# Autodesk Inventor assembly: Assembly_final
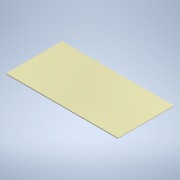
[picture p0: Inventor's stored thumbnail of the model, 180x180]
Saved by Autodesk Inventor 2021 (Build 250183000, 183)
## iProperties
Created: 2021-02-05
Part Number: Assembly_final
Document SubType Name: Assembly
Designer: User
Author: User
## Documents named in this file (3)
- C:\Users\User\Documents\GitHub\2020-srw-rc-car\CoilDesign\CAD Track\Assembly_final.iam
- C:\Users\User\Documents\GitHub\2020-srw-rc-car\CoilDesign\CAD Track\CoilLayer\wire_holder_lasercutting800.ipt
- C:\Users\User\Documents\GitHub\2020-srw-rc-car\CoilDesign\CAD Track\Top Layer\TopCoverLayerNew.ipt
## Components (2 placed, 2 different names)
1. wire_holder_lasercutting800:1 — Rigid:1
2. TopCoverLayerNew:1 — Rigid:1
## Relationships (1: WeldJoint 1)
- Rigid:1 [WeldJoint]: wire_holder_lasercutting800:1 ↔ TopCoverLayerNew:1
